# Autodesk Inventor assembly: Montagem
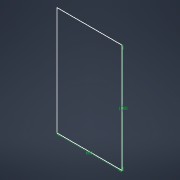
[picture p0: Inventor's stored thumbnail of the model, 180x180]
Saved by Autodesk Inventor 2022 (Build 260153000, 153)
## iProperties
Created: 2022-05-21
Part Number: Montagem
Document SubType Name: Assembly
Designer: Gugarauj07
Author: Gugarauj07
## Documents named in this file (2)
- C:\Users\Gugarauj07\PycharmProjects\Eletronica_2022\CADS\Carrinho_Rolima\Montagem.iam
- C:\Users\Gugarauj07\PycharmProjects\Eletronica_2022\CADS\Carrinho_Rolima\Base.ipt
## Components (1 placed, 1 different names)
1. Base:1 — Coincidente:1, Coincidente:2, Coincidente:3
## Relationships (3: Mate 3)
- Coincidente:1 [Mate]: Base:1
- Coincidente:2 [Mate]: Base:1
- Coincidente:3 [Mate]: Base:1
